# Autodesk Inventor assembly: finger
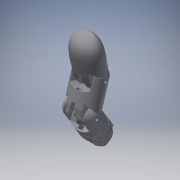
[picture p0: Inventor's stored thumbnail of the model, 180x180]
Saved by Autodesk Inventor 2019 (Build 230136000, 136)
## iProperties
Created: 2016-03-08
Part Number: finger
Document SubType Name: Assembly
Designer: Marco Prata
Mass: 0.0261856 g
Surface Area: 59.2097 cm^2
Volume: 0.0261856 cm^3
Density: 1 g/cm^3
## Documents named in this file (3)
- Z:\Nico_N\NICO-CAD-master\NICO_CAD_master\hand\Seed Finger\finger.iam
- Z:\Nico_N\NICO-CAD-master\NICO_CAD_master\hand\Seed Finger\fingertip.ipt
- Z:\Nico_N\NICO-CAD-master\NICO_CAD_master\hand\Seed Finger\finger_segment.ipt
## Components (3 placed, 2 different names)
1. finger_segment:1 — Insert:1, Insert:2
2. finger_segment:2 — Insert:2
3. fingertip:1 — Insert:1
## Relationships (2: Insert 2)
- Insert:1 (0.5 mm): finger_segment:1 ↔ fingertip:1
- Insert:2 (0.5 mm): finger_segment:1 ↔ finger_segment:2
